# Autodesk Inventor assembly: アセンブリ1
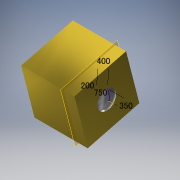
[picture p0: Inventor's stored thumbnail of the model, 180x180]
Saved by Autodesk Inventor 2019.1 (Build 231200000, 200)
## iProperties
Created: 2018-12-21
Part Number: アセンブリ1
Material: 一般
Document SubType Name: Assembly
Designer: Masaya
Author: Masaya
## Documents named in this file (3)
- C:\Users\Masaya\Documents\航空宇宙\卒業設計\seed_bank_in_space\cad\アセンブリ1.iam
- C:\Users\Masaya\Documents\航空宇宙\卒業設計\seed_bank_in_space\cad\hako.ipt
- C:\Users\Masaya\Documents\航空宇宙\卒業設計\seed_bank_in_space\cad\capcule.ipt
## Components (2 placed, 2 different names)
1. hako:1 — メイト:1, 正接:1
2. capcule:1 — メイト:1, 正接:1
## Relationships (2: Mate 1, Tangent 1)
- メイト:1 [Mate]: hako:1 ↔ capcule:1
- 正接:1 [Tangent]: hako:1 ↔ capcule:1
